# Autodesk Inventor assembly: Robot Chassis 2014 Railgun
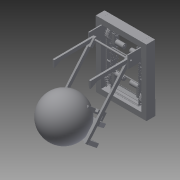
[picture p0: Inventor's stored thumbnail of the model, 180x180]
Saved by Autodesk Inventor 2014 (Build 180170000, 170)
## iProperties
Created: 2014-01-08
Part Number: Robot Chassis 2014 Railgun
Document SubType Name: Assembly
Designer: 300593
Translation Standard: STEP AP203
FileName: AM14U Long and AM14U Wide.STEP
PreProcessor: SolidWorks 2010
PostProcessor: Build: 138, Release: 2013 RTM - Date: Thu 03/01/2012
Sent Units: inch
Uncertainty: 1e-05
Author: 300593
## Documents named in this file (14)
- H:\Robotics\FRC\2014\CAD\Frame\Robot Chassis 2014 Railgun.iam
- G:\CAD\Frame\AM14U Long.iam
- G:\CAD\Frame\Left-6-inch-HD-Mecanum-Wheel.iam
- G:\CAD\Frame\Right-6-inch-HD-Mecanum-Wheel.iam
- G:\CAD\Frame\Toughbox-nano-hex-asm.iam
- G:\CAD\Additions\BumperFront.ipt
- G:\CAD\Additions\BumperSide.ipt
- G:\CAD\Additions\Ball.ipt
- G:\CAD\Frame\armholder.ipt
- G:\CAD\Frame\armcylinder.ipt
- G:\CAD\Frame\armthatworks.ipt
- G:\CAD\Frame\rail.ipt
- G:\CAD\Frame\railrider.ipt
- C:\Users\zachary\Documents\tension holder.ipt
## Components (23 placed, 13 different names)
1. AM14U Long:1 [sub-assembly] — Mate:1, Mate:2, Mate:3, Mate:4, Mate:5, Mate:6, Mate:7, Mate:8, Mate:9, Mate:10, Mate:11, Mate:12, Mate:17, Mate:18, Mate:19, Mate:20, Flush:1, Flush:3, Flush:5, Mate:22, Mate:24, Mate:29
2. Left-6-inch-HD-Mecanum-Wheel:1 [sub-assembly] — Mate:16, Mate:17
3. Left-6-inch-HD-Mecanum-Wheel:2 [sub-assembly] — Mate:14, Mate:20
4. Right-6-inch-HD-Mecanum-Wheel:1 [sub-assembly] — Mate:13, Mate:19
5. Right-6-inch-HD-Mecanum-Wheel:2 [sub-assembly] — Mate:15, Mate:18
6. Toughbox-nano-hex-asm:1 [sub-assembly] — Mate:7, Mate:10, Mate:12, Mate:13
7. Toughbox-nano-hex-asm:2 [sub-assembly] — Mate:8, Mate:9, Mate:11, Mate:14
8. Toughbox-nano-hex-asm:3 [sub-assembly] — Mate:4, Mate:5, Mate:6, Mate:15
9. Toughbox-nano-hex-asm:4 [sub-assembly] — Mate:1, Mate:2, Mate:3, Mate:16
10. BumperFront:1 — Flush:1, Flush:3, Flush:5, Flush:6, Flush:7, Flush:8, Flush:10, Flush:15, Mate:25, Mate:28
11. BumperSide:1 — Flush:6, Flush:10, Flush:15, Flush:16, Flush:17, Mate:23, Mate:27
12. BumperSide:2 — Mate:22, Flush:7, Flush:8, Mate:26
13. BumperFront:2 — Flush:16, Flush:17, Mate:23
14. Ball:1
15. armholder:1 — Mate:24, Mate:25, Mate:26, Mate:30, Mate:33
16. armholder:2 — Mate:27, Mate:28, Mate:29, Flush:18, Flush:19
17. armcylinder:1 — Flush:18, Mate:30, Mate:31, Mate:32, Mate:34, Mate:37
18. armthatworks:1 — Flush:19, Mate:31, Flush:20, Mate:35
19. armthatworks:2 — Mate:32, Mate:33, Flush:20, Mate:36
20. rail:1 — Mate:34, Mate:35, Flush:21, Flush:22, Mate:38
21. rail:2 — Mate:36, Mate:37, Flush:21, Flush:23, Flush:24, Flush:25, Flush:26
22. railrider:1 — Flush:22, Flush:23
23. tension holder:1 — Flush:24, Mate:38, Flush:25, Flush:26
## Relationships (56: Mate 37, Flush 19)
- Mate:1: AM14U Long:1 ↔ Toughbox-nano-hex-asm:4
- Mate:2: AM14U Long:1 ↔ Toughbox-nano-hex-asm:4
- Mate:3: AM14U Long:1 ↔ Toughbox-nano-hex-asm:4
- Mate:4: AM14U Long:1 ↔ Toughbox-nano-hex-asm:3
- Mate:5: AM14U Long:1 ↔ Toughbox-nano-hex-asm:3
- Mate:6: AM14U Long:1 ↔ Toughbox-nano-hex-asm:3
- Mate:7: AM14U Long:1 ↔ Toughbox-nano-hex-asm:1
- Mate:8: AM14U Long:1 ↔ Toughbox-nano-hex-asm:2
- Mate:9: AM14U Long:1 ↔ Toughbox-nano-hex-asm:2
- Mate:10: AM14U Long:1 ↔ Toughbox-nano-hex-asm:1
- Mate:11: AM14U Long:1 ↔ Toughbox-nano-hex-asm:2
- Mate:12: AM14U Long:1 ↔ Toughbox-nano-hex-asm:1
- Mate:13: Right-6-inch-HD-Mecanum-Wheel:1 ↔ Toughbox-nano-hex-asm:1
- Mate:14: Left-6-inch-HD-Mecanum-Wheel:2 ↔ Toughbox-nano-hex-asm:2
- Mate:15: Right-6-inch-HD-Mecanum-Wheel:2 ↔ Toughbox-nano-hex-asm:3
- Mate:16: Left-6-inch-HD-Mecanum-Wheel:1 ↔ Toughbox-nano-hex-asm:4
- Mate:17 (19.3294 mm): AM14U Long:1 ↔ Left-6-inch-HD-Mecanum-Wheel:1
- Mate:18 (19.3294 mm): AM14U Long:1 ↔ Right-6-inch-HD-Mecanum-Wheel:2
- Mate:19 (19.3294 mm): AM14U Long:1 ↔ Right-6-inch-HD-Mecanum-Wheel:1
- Mate:20 (19.3294 mm): AM14U Long:1 ↔ Left-6-inch-HD-Mecanum-Wheel:2
- Flush:1: AM14U Long:1 ↔ BumperFront:1
- Flush:3: AM14U Long:1 ↔ BumperFront:1
- Flush:5 (-48.3362 mm): AM14U Long:1 ↔ BumperFront:1
- Flush:6: BumperFront:1 ↔ BumperSide:1
- Mate:22: AM14U Long:1 ↔ BumperSide:2
- Flush:7: BumperFront:1 ↔ BumperSide:2
- Flush:8: BumperFront:1 ↔ BumperSide:2
- Flush:10: BumperFront:1 ↔ BumperSide:1
- Flush:15: BumperFront:1 ↔ BumperSide:1
- Flush:16: BumperSide:1 ↔ BumperFront:2
- Flush:17: BumperSide:1 ↔ BumperFront:2
- Mate:23: BumperSide:1 ↔ BumperFront:2
- Mate:24: AM14U Long:1 ↔ armholder:1
- Mate:25: BumperFront:1 ↔ armholder:1
- Mate:26: BumperSide:2 ↔ armholder:1
- Mate:27: BumperSide:1 ↔ armholder:2
- Mate:28: BumperFront:1 ↔ armholder:2
- Mate:29: AM14U Long:1 ↔ armholder:2
- Flush:18: armholder:2 ↔ armcylinder:1
- Mate:30: armholder:1 ↔ armcylinder:1
- Flush:19: armholder:2 ↔ armthatworks:1
- Mate:31: armcylinder:1 ↔ armthatworks:1
- Mate:32: armcylinder:1 ↔ armthatworks:2
- Mate:33: armholder:1 ↔ armthatworks:2
- Flush:20: armthatworks:1 ↔ armthatworks:2
- Mate:34: armcylinder:1 ↔ rail:1
- Mate:35: armthatworks:1 ↔ rail:1
- Mate:36: armthatworks:2 ↔ rail:2
- Mate:37: armcylinder:1 ↔ rail:2
- Flush:21: rail:1 ↔ rail:2
- Flush:22: rail:1 ↔ railrider:1
- Flush:23: rail:2 ↔ railrider:1
- Flush:24: rail:2 ↔ tension holder:1
- Mate:38: rail:1 ↔ tension holder:1
- Flush:25: rail:2 ↔ tension holder:1
- Flush:26 (-25.4 mm): rail:2 ↔ tension holder:1
